# Autodesk Inventor assembly: Zusammenbau_DruckLuftMotor
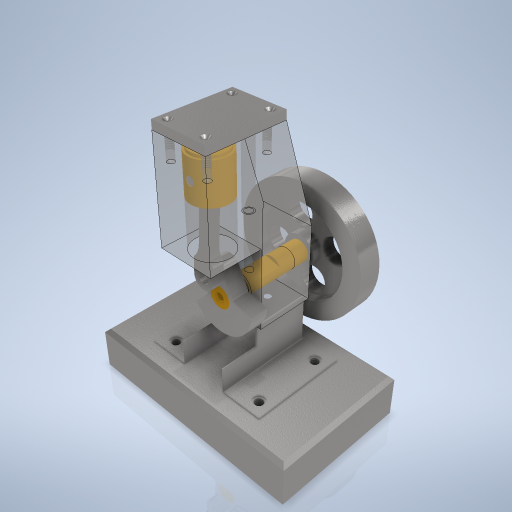
[picture p0: Inventor's stored thumbnail of the model, 512x512]
Saved by Autodesk Inventor 2024.2 (Build 282272000, 272)
## iProperties
Created: 2024-01-15
Part Number: Zusammenbau_DruckLuftMotor
Document SubType Name: Assembly
Designer: ffogue
Author: ffogue
## Documents named in this file (11)
- C:\Users\Fabri\Documents\Inventor\Motor\Zusammenbau_DruckLuftMotor.iam
- C:\Users\Fabri\Documents\Inventor\Motor\Grundplatte.ipt
- C:\Users\Fabri\Documents\Inventor\Motor\Bügelbefestigung.ipt
- C:\Users\Fabri\Documents\Inventor\Motor\Kolben.ipt
- C:\Users\Fabri\Documents\Inventor\Motor\Pleuel.ipt
- C:\Users\Fabri\Documents\Inventor\Motor\Kurbelzapfen.ipt
- C:\Users\Fabri\Documents\Inventor\Motor\Schwungscheibe.ipt
- C:\Users\Fabri\Documents\Inventor\Motor\Kurbel.ipt
- C:\Users\Fabri\Documents\Inventor\Motor\MotorBlock.ipt
- C:\Users\Fabri\Documents\Inventor\Motor\Kurbelwelle.ipt
- C:\Users\Fabri\Documents\Inventor\Motor\Zylinderkopf.ipt
## Components (10 placed, 10 different names)
1. Bügelbefestigung:1 — Einfügen:1, Winkel:1, Einfügen:2, Winkel:2
2. Pleuel:1 — Einfügen:3, Einfügen:7
3. Kurbelzapfen:1 — Einfügen:3, Drehbar:1
4. Kolben:1 — Zylindrisch:1, Drehbar:1, Passend:5
5. MotorBlock:1 — Einfügen:2, Winkel:2, Zylindrisch:1, Passend:2, Passend:4, Einfügen:10, Fluchtend:1
6. Kurbel:1 — Einfügen:7, Winkel:6, Einfügen:8, Winkel:7
7. Grundplatte:1 — Einfügen:1, Winkel:1
8. Schwungscheibe:1 — Motion, Winkel:6, Einfügen:9
9. Kurbelwelle:1 — Einfügen:8, Winkel:7, Einfügen:9, Passend:1
10. Zylinderkopf:1 — Einfügen:10, Fluchtend:1
## Relationships (21: Insert 7, Mate 6, Angle 5, CylindricalJoint 1, RevoluteJoint 1, Flush 1)
- Einfügen:1 [Insert]: Bügelbefestigung:1 ↔ Grundplatte:1
- Winkel:1 [Angle] (270 deg): Bügelbefestigung:1 ↔ Grundplatte:1
- Einfügen:2 [Insert]: Bügelbefestigung:1 ↔ MotorBlock:1
- Winkel:2 [Angle] (0 deg): Bügelbefestigung:1 ↔ MotorBlock:1
- Einfügen:3 [Insert] (-8.8 mm): Pleuel:1 ↔ Kurbelzapfen:1
- Zylindrisch:1 [CylindricalJoint]: Kolben:1 ↔ MotorBlock:1
- Drehbar:1 [RevoluteJoint] (-13.8 mm): Kurbelzapfen:1 ↔ Kolben:1
- Motion [Angle] (1424 deg): Schwungscheibe:1
- Einfügen:7 [Insert]: Pleuel:1 ↔ Kurbel:1
- Winkel:6 [Angle] (300 deg): Kurbel:1 ↔ Schwungscheibe:1
- Einfügen:8 [Insert] (-34 mm): Kurbel:1 ↔ Kurbelwelle:1
- Winkel:7 [Angle] (0 deg): Kurbel:1 ↔ Kurbelwelle:1
- Einfügen:9 [Insert]: Schwungscheibe:1 ↔ Kurbelwelle:1
- Passend:1 [Mate]: Kurbelwelle:1
- Passend:2 [Mate]: MotorBlock:1
- Passend:3 [Mate]
- Passend:4 [Mate]: MotorBlock:1
- Passend:5 [Mate]: Kolben:1
- Passend:6 [Mate]
- Einfügen:10 [Insert]: MotorBlock:1 ↔ Zylinderkopf:1
- Fluchtend:1 [Flush]: MotorBlock:1 ↔ Zylinderkopf:1
